# Autodesk Inventor assembly: ASY GBK 1320 long wall shield 5
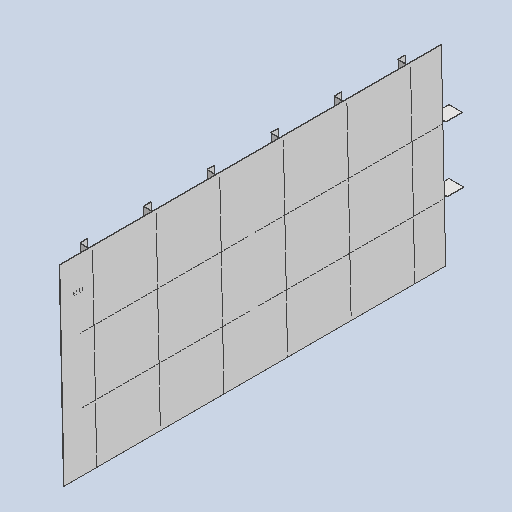
[picture p0: Inventor's stored thumbnail of the model, 512x512]
Saved by Autodesk Inventor 2026.3 (Build 303398000, 398)
## iProperties
Created: 2026-05-07
Part Number: ASY GBK 1320 long wall shield 5
Document SubType Name: Assembly
Designer: pokla
Mass: 215512 g
Surface Area: 139105 cm^2
Volume: 27453.8 cm^3
Density: 7.85 g/cm^3
Stock Number: 1320
Author: admin
## Documents named in this file (6)
- C:\Users\admin\Documents\Inventor\GBK-Gubkinskiy\ASY GBK 1320 long wall shield 5.iam
- C:\Users\admin\Documents\Inventor\GBK-Gubkinskiy\GBK 0101 main rib.ipt
- C:\Users\admin\Documents\Inventor\GBK-Gubkinskiy\GBK 0302 stringer 7.ipt
- C:\Users\admin\Documents\Inventor\GBK-Gubkinskiy\GBK 0303 stringer 8.ipt
- C:\Users\admin\Documents\Inventor\GBK-Gubkinskiy\GBK 0301 third rib.ipt
- C:\Users\admin\Documents\Inventor\GBK-Gubkinskiy\GBK 1325 shield 1.2.ipt
## Components (11 placed, 4 different names)
1. GBK 0302 stringer 7:1 — Rigid:4
2. GBK 0303 stringer 8:1 — Rigid:3, Mate:2, Flush:2
3. GBK 0303 stringer 8:2 — Rigid:3
4. GBK 0302 stringer 7:2 — Rigid:4
5. GBK 1325 shield 1.2:1 — Mate:3, Flush:1, Mate:4, Flush:2
6. GBK 0301 third rib:1 — Mate:1, Mate:3
7. GBK 0301 third rib:2
8. GBK 0301 third rib:3
9. GBK 0301 third rib:4
10. GBK 0301 third rib:5
11. GBK 0301 third rib:6
## Component patterns: (6 elements, first: GBK 0301 third rib:1)
## Relationships (10: WeldJoint 4, Mate 4, Flush 2)
- [WeldJoint] (4 mm): GBK 0302 stringer 7:1 ↔ GBK 0301 third rib:1
- [WeldJoint] (4 mm): GBK 0303 stringer 8:1 ↔ GBK 0301 third rib:1
- Rigid:3 [WeldJoint] (1 mm): GBK 0303 stringer 8:1 ↔ GBK 0303 stringer 8:2
- Rigid:4 [WeldJoint] (1 mm): GBK 0302 stringer 7:1 ↔ GBK 0302 stringer 7:2
- Mate:1: GBK 0301 third rib:1
- Mate:2: GBK 0303 stringer 8:1
- Mate:3: GBK 1325 shield 1.2:1 ↔ GBK 0301 third rib:1
- Flush:1: GBK 1325 shield 1.2:1
- Mate:4: GBK 1325 shield 1.2:1
- Flush:2 (155 mm): GBK 0303 stringer 8:1 ↔ GBK 1325 shield 1.2:1
## Named parameters: Шаг_шпангоутов = 496.66667 mm
